# Autodesk Inventor assembly: FY 15 FM
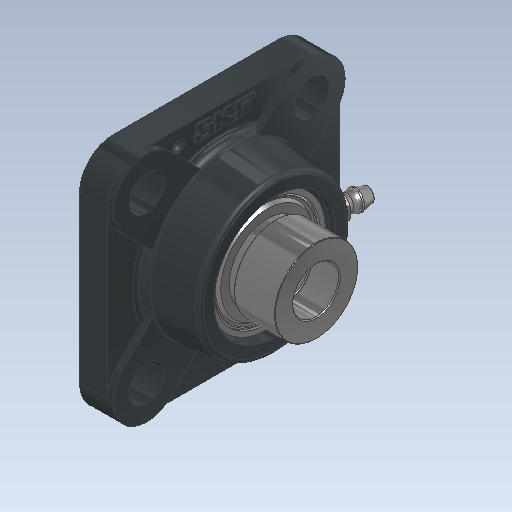
[picture p0: Inventor's stored thumbnail of the model, 512x512]
Saved by Autodesk Inventor 2020 (Build 240168000, 168)
## iProperties
Part Number: FY 15 FM
Catalog Web Link: www.cadenas.de
Description: AYF_001HC_HH_HY-Y-bearing square flanged units
Vendor: SKF
Document SubType Name: Assembly
Designer: partserver
Manufacturer: SKF
Mass: 400 g
Surface Area: 332.088 cm^2
Volume: 55.8847 cm^3
Density: 7.1576 g/cm^3
Category: PARTsolutions
Company: SKF
PSOL_IDENT_0: {$CADENAS_DATA\23d-libs\skf\bearings_units_and_housings\bearing_units\ball_bearing_units\y-units\ayf
PSOL_IDENT_1: _001hc_hh_hy.prj},187 {VTYP=3D},{STYP=ASSTAB},{NB=FY 15 FM},{LINA=FY 15 FM},{NN=AYF_001HC_HH_HY},{DA
PSOL_IDENT_2: TE=20.08.2020 12:22:38},{GEOMDATE=20.08.2020 12:22:32},{VERSION=},{LINEID=52770},{WBVAR=COVER},{WBNU
PSOL_IDENT_3: MERIC=}  {NB=FY 15 FM},{LINA=FY 15 FM},{KT=DUMMY},{DESIGNATION=FY 15 FM},{HOUSING=FY 503 M},{BEARING=
PSOL_IDENT_4: YET 203/15},{COVER=},{DD=15},{DDX=},{DDALG=15.000},{DD1=24.200},{DD2=27.200},{DD3=},{AALG=26.000},{A=
PSOL_IDENT_5: 26},{AX=},{AXX=},{A1ALG=11.000},{A1=11},{A1X=},{A1XX=},{A3ALG=3.200},{A3=3.2},{A3X=},{A5ALG=0.000},{
PSOL_IDENT_6: A5=},{A5X=},{A5XX=},{B=MIN},{B1=28.600},{B1X=},{B4ALG=4.750},{B4=},{B4X=4.75},{DAAALG=55.600},{DAA=5
PSOL_IDENT_7: 5.6},{DAAX=},{DB=MIN},{DB1=50.000},{DB1X=},{DB2=53.000},{DB2X=},{HA=},{J=54.000},{JX=},{JXX=},{L=76.
PSOL_IDENT_8: 000},{LX=},{LXX=},{N=11.500},{NX=},{NXX=},{SS1=22.100},{SS1X=},{T=39.600},{TX=},{DN=6.500},{SWN=7},{
PSOL_IDENT_9: GN=1/4-28 SAE-LT},{RG=1/4-28 UNF},{RGX=},{R1=19},{R1X=},{J6=66},{J7=14.500},{N4=4},{D=40.000},{C=12.
PSOL_IDENT_10: 000},{R12=0.300},{DW=6.747},{B3=13.500},{PITCH=28.500},{LOAD1=9.560},{LOAD2=4.750},{LOAD3=0.200},{SP
PSOL_IDENT_11: EED1=9500},{II=1},{Z=8},{MASS=0.400},{MASSX=},{G2=M6x0.75},{HKSGS=3},{RTTGS=4},{ALPHA=},{GALG=10.000
PSOL_IDENT_12: },{G=10},{GX=},{GXX=},{GINALG=0.375},{GIN=0.375000002475},{GINX=},{GINXX=},{EC=},{BS=},{SLEEVE=},{PO
PSOL_IDENT_13: PULAR=},{D1=MIN},{K=1.3},{CC1=3.6},{BRGTYP=BBY_005},{COVERALG=  '', 'No end cover' },{SUPPRESSED=uns
PSOL_IDENT_14: uppressed},{TC=FY 15 FM},{PPATH=y-bearing_square_flanged_units_parts/ayf_001hc_hh_hy_asmtpl.prj}
NB: FY 15 FM
NN: AYF_001HC_HH_HY
NT: Y-bearing square flanged units
NBSYN: $TC.
LINA: FY 15 FM
CATALOG: SKF
DESIGNATION: FY 15 FM
HOUSING: FY 503 M
BEARING: YET 203/15
COVER: No end cover
DDALG: 15
J: 54
L: 76
T: 39.6
LOAD1: 9.56
LOAD2: 4.75
SPEED1: 9500
SUPPLIER: SKF
ARTICLENO: FY 15 FM
BOMINFO: FY 15 FM
CREATOR: CADENAS GmbH
Title: FY 15 FM
Author: Cadenas PARTsolutions
Comments: Y-bearing square flanged units
## Documents named in this file (6)
- C:\Users\Hesekiel\Desktop\Equatorial-Mount-MUM\Mechanika\Mechanizm elewacji Filip\CAD\FY 15 FM\FY 15 FM.iam
- C:\Users\Hesekiel\Desktop\Equatorial-Mount-MUM\Mechanika\Mechanizm elewacji Filip\CAD\FY 15 FM\FY 15 FM0_375000002475-dummy.ipt
- C:\Users\Hesekiel\Desktop\Equatorial-Mount-MUM\Mechanika\Mechanizm elewacji Filip\CAD\FY 15 FM\FY 503 M-housing.ipt
- C:\Users\Hesekiel\Desktop\Equatorial-Mount-MUM\Mechanika\Mechanizm elewacji Filip\CAD\FY 15 FM\1_4-28 SAE-LT.ipt
- C:\Users\Hesekiel\Desktop\Equatorial-Mount-MUM\Mechanika\Mechanizm elewacji Filip\CAD\FY 15 FM\YET 203_15-24_21030112021228_6-bearing.ipt
- C:\Users\Hesekiel\Desktop\Equatorial-Mount-MUM\Mechanika\Mechanizm elewacji Filip\CAD\FY 15 FM\15-40-19_1-12-ybrg2-124-6_747-28_5.ipt
## Components (12 placed, 5 different names)
1. FY 15 FM0_375000002475-dummy:1 — brg_XY@1 <-> housing_XY@2, brg_Z@1 <-> housing_Z@2, brg_YZ@1 <-> housing_YZ@2
2. FY 503 M-housing:1 — brg_XY@1 <-> housing_XY@2, brg_Z@1 <-> housing_Z@2, brg_YZ@1 <-> housing_YZ@2, gn_XY@2 <-> gn_XY@3, gn_Z@2 <-> gn_Z@3, gn_YZ@2 <-> gn_YZ@3, housing_XY@2 <-> brg3_XY@4, housing_Z@2 <-> brg3_Z@4, housing_YZ@2 <-> brg3_YZ@4
3. 1_4-28 SAE-LT:1 — gn_XY@2 <-> gn_XY@3, gn_Z@2 <-> gn_Z@3, gn_YZ@2 <-> gn_YZ@3
4. YET 203_15-24_21030112021228_6-bearing:1 — housing_XY@2 <-> brg3_XY@4, housing_Z@2 <-> brg3_Z@4, housing_YZ@2 <-> brg3_YZ@4, ball_1_XY@4 <-> ball_XY@5, ball_1_Z@4 <-> ball_Z@5, ball_1_YZ@4 <-> ball_YZ@5, ball_2_XY@4 <-> ball_XY@6, ball_2_Z@4 <-> ball_Z@6, ball_2_YZ@4 <-> ball_YZ@6, ball_3_XY@4 <-> ball_XY@7, ball_3_Z@4 <-> ball_Z@7, ball_3_YZ@4 <-> ball_YZ@7, ball_4_XY@4 <-> ball_XY@8, ball_4_Z@4 <-> ball_Z@8, ball_4_YZ@4 <-> ball_YZ@8, ball_5_XY@4 <-> ball_XY@9, ball_5_Z@4 <-> ball_Z@9, ball_5_YZ@4 <-> ball_YZ@9, ball_6_XY@4 <-> ball_XY@10, ball_6_Z@4 <-> ball_Z@10, ball_6_YZ@4 <-> ball_YZ@10, ball_7_XY@4 <-> ball_XY@11, ball_7_Z@4 <-> ball_Z@11, ball_7_YZ@4 <-> ball_YZ@11, ball_8_XY@4 <-> ball_XY@12, ball_8_Z@4 <-> ball_Z@12, ball_8_YZ@4 <-> ball_YZ@12
5. 15-40-19_1-12-ybrg2-124-6_747-28_5:1 — ball_1_XY@4 <-> ball_XY@5, ball_1_Z@4 <-> ball_Z@5, ball_1_YZ@4 <-> ball_YZ@5
6. 15-40-19_1-12-ybrg2-124-6_747-28_5:2 — ball_2_XY@4 <-> ball_XY@6, ball_2_Z@4 <-> ball_Z@6, ball_2_YZ@4 <-> ball_YZ@6
7. 15-40-19_1-12-ybrg2-124-6_747-28_5:3 — ball_3_XY@4 <-> ball_XY@7, ball_3_Z@4 <-> ball_Z@7, ball_3_YZ@4 <-> ball_YZ@7
8. 15-40-19_1-12-ybrg2-124-6_747-28_5:4 — ball_4_XY@4 <-> ball_XY@8, ball_4_Z@4 <-> ball_Z@8, ball_4_YZ@4 <-> ball_YZ@8
9. 15-40-19_1-12-ybrg2-124-6_747-28_5:5 — ball_5_XY@4 <-> ball_XY@9, ball_5_Z@4 <-> ball_Z@9, ball_5_YZ@4 <-> ball_YZ@9
10. 15-40-19_1-12-ybrg2-124-6_747-28_5:6 — ball_6_XY@4 <-> ball_XY@10, ball_6_Z@4 <-> ball_Z@10, ball_6_YZ@4 <-> ball_YZ@10
11. 15-40-19_1-12-ybrg2-124-6_747-28_5:7 — ball_7_XY@4 <-> ball_XY@11, ball_7_Z@4 <-> ball_Z@11, ball_7_YZ@4 <-> ball_YZ@11
12. 15-40-19_1-12-ybrg2-124-6_747-28_5:8 — ball_8_XY@4 <-> ball_XY@12, ball_8_Z@4 <-> ball_Z@12, ball_8_YZ@4 <-> ball_YZ@12
## Relationships (33: Mate 21, Angle 11, Flush 1)
- brg_XY@1 <-> housing_XY@2 [Mate]: FY 15 FM0_375000002475-dummy:1 ↔ FY 503 M-housing:1
- brg_Z@1 <-> housing_Z@2 [Mate]: FY 15 FM0_375000002475-dummy:1 ↔ FY 503 M-housing:1
- brg_YZ@1 <-> housing_YZ@2 [Angle] (180 deg): FY 15 FM0_375000002475-dummy:1 ↔ FY 503 M-housing:1
- gn_XY@2 <-> gn_XY@3 [Mate]: FY 503 M-housing:1 ↔ 1_4-28 SAE-LT:1
- gn_Z@2 <-> gn_Z@3 [Mate]: FY 503 M-housing:1 ↔ 1_4-28 SAE-LT:1
- gn_YZ@2 <-> gn_YZ@3 [Angle] (0 deg): FY 503 M-housing:1 ↔ 1_4-28 SAE-LT:1
- housing_XY@2 <-> brg3_XY@4 [Flush] (39.6 mm): FY 503 M-housing:1 ↔ YET 203_15-24_21030112021228_6-bearing:1
- housing_Z@2 <-> brg3_Z@4 [Mate]: FY 503 M-housing:1 ↔ YET 203_15-24_21030112021228_6-bearing:1
- housing_YZ@2 <-> brg3_YZ@4 [Angle] (0 deg): FY 503 M-housing:1 ↔ YET 203_15-24_21030112021228_6-bearing:1
- ball_1_XY@4 <-> ball_XY@5 [Mate]: YET 203_15-24_21030112021228_6-bearing:1 ↔ 15-40-19_1-12-ybrg2-124-6_747-28_5:1
- ball_1_Z@4 <-> ball_Z@5 [Mate]: YET 203_15-24_21030112021228_6-bearing:1 ↔ 15-40-19_1-12-ybrg2-124-6_747-28_5:1
- ball_1_YZ@4 <-> ball_YZ@5 [Angle] (0 deg): YET 203_15-24_21030112021228_6-bearing:1 ↔ 15-40-19_1-12-ybrg2-124-6_747-28_5:1
- ball_2_XY@4 <-> ball_XY@6 [Mate]: YET 203_15-24_21030112021228_6-bearing:1 ↔ 15-40-19_1-12-ybrg2-124-6_747-28_5:2
- ball_2_Z@4 <-> ball_Z@6 [Mate]: YET 203_15-24_21030112021228_6-bearing:1 ↔ 15-40-19_1-12-ybrg2-124-6_747-28_5:2
- ball_2_YZ@4 <-> ball_YZ@6 [Angle] (0 deg): YET 203_15-24_21030112021228_6-bearing:1 ↔ 15-40-19_1-12-ybrg2-124-6_747-28_5:2
- ball_3_XY@4 <-> ball_XY@7 [Mate]: YET 203_15-24_21030112021228_6-bearing:1 ↔ 15-40-19_1-12-ybrg2-124-6_747-28_5:3
- ball_3_Z@4 <-> ball_Z@7 [Mate]: YET 203_15-24_21030112021228_6-bearing:1 ↔ 15-40-19_1-12-ybrg2-124-6_747-28_5:3
- ball_3_YZ@4 <-> ball_YZ@7 [Angle] (0 deg): YET 203_15-24_21030112021228_6-bearing:1 ↔ 15-40-19_1-12-ybrg2-124-6_747-28_5:3
- ball_4_XY@4 <-> ball_XY@8 [Mate]: YET 203_15-24_21030112021228_6-bearing:1 ↔ 15-40-19_1-12-ybrg2-124-6_747-28_5:4
- ball_4_Z@4 <-> ball_Z@8 [Mate]: YET 203_15-24_21030112021228_6-bearing:1 ↔ 15-40-19_1-12-ybrg2-124-6_747-28_5:4
- ball_4_YZ@4 <-> ball_YZ@8 [Angle] (0 deg): YET 203_15-24_21030112021228_6-bearing:1 ↔ 15-40-19_1-12-ybrg2-124-6_747-28_5:4
- ball_5_XY@4 <-> ball_XY@9 [Mate]: YET 203_15-24_21030112021228_6-bearing:1 ↔ 15-40-19_1-12-ybrg2-124-6_747-28_5:5
- ball_5_Z@4 <-> ball_Z@9 [Mate]: YET 203_15-24_21030112021228_6-bearing:1 ↔ 15-40-19_1-12-ybrg2-124-6_747-28_5:5
- ball_5_YZ@4 <-> ball_YZ@9 [Angle] (0 deg): YET 203_15-24_21030112021228_6-bearing:1 ↔ 15-40-19_1-12-ybrg2-124-6_747-28_5:5
- ball_6_XY@4 <-> ball_XY@10 [Mate]: YET 203_15-24_21030112021228_6-bearing:1 ↔ 15-40-19_1-12-ybrg2-124-6_747-28_5:6
- ball_6_Z@4 <-> ball_Z@10 [Mate]: YET 203_15-24_21030112021228_6-bearing:1 ↔ 15-40-19_1-12-ybrg2-124-6_747-28_5:6
- ball_6_YZ@4 <-> ball_YZ@10 [Angle] (0 deg): YET 203_15-24_21030112021228_6-bearing:1 ↔ 15-40-19_1-12-ybrg2-124-6_747-28_5:6
- ball_7_XY@4 <-> ball_XY@11 [Mate]: YET 203_15-24_21030112021228_6-bearing:1 ↔ 15-40-19_1-12-ybrg2-124-6_747-28_5:7
- ball_7_Z@4 <-> ball_Z@11 [Mate]: YET 203_15-24_21030112021228_6-bearing:1 ↔ 15-40-19_1-12-ybrg2-124-6_747-28_5:7
- ball_7_YZ@4 <-> ball_YZ@11 [Angle] (0 deg): YET 203_15-24_21030112021228_6-bearing:1 ↔ 15-40-19_1-12-ybrg2-124-6_747-28_5:7
- ball_8_XY@4 <-> ball_XY@12 [Mate]: YET 203_15-24_21030112021228_6-bearing:1 ↔ 15-40-19_1-12-ybrg2-124-6_747-28_5:8
- ball_8_Z@4 <-> ball_Z@12 [Mate]: YET 203_15-24_21030112021228_6-bearing:1 ↔ 15-40-19_1-12-ybrg2-124-6_747-28_5:8
- ball_8_YZ@4 <-> ball_YZ@12 [Angle] (0 deg): YET 203_15-24_21030112021228_6-bearing:1 ↔ 15-40-19_1-12-ybrg2-124-6_747-28_5:8
